# Autodesk Inventor assembly: XRevit Filter column D1200
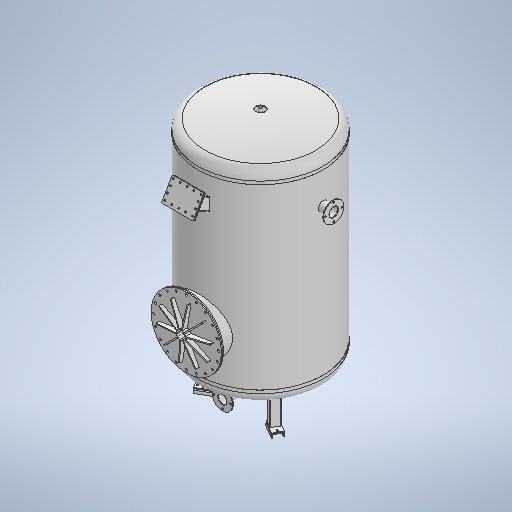
[picture p0: Inventor's stored thumbnail of the model, 512x512]
Saved by Autodesk Inventor 2025.4 (Build 294407000, 407)
## iProperties
Created: 2025-02-13
Part Number: XRevit Filter column D1200
Document SubType Name: Assembly
Designer: pokla
Mass: 483166 g
Surface Area: 236267 cm^2
Volume: 67816.7 cm^3
Density: 7.1246 g/cm^3
allow_slope_adjustment: 0 ul
flow_configuration2: 1 ul
flow_direction: 2 ul
loss_method: 0 ul
radius: 45,500 mm
radius: 16,750 mm
Author: pokla
Revision Number: 3
## Documents named in this file (23)
- C:\Users\pokla\Documents\Inventor\PRS-Purovskii\Model\PRS-filter 1200\ASY PRS Filter column D1200.iam
- C:\Users\pokla\Documents\Inventor\PRS-Purovskii\Model\PRS-filter 1200\PRS 1200-22 accses hatch flangeipt.ipt
- C:\Users\pokla\Documents\Inventor\PRS-Purovskii\Model\PRS-filter 1200\PRS 1200-11 accses hatch tube.ipt
- C:\Users\pokla\Documents\Inventor\PRS-Purovskii\Model\PRS-filter 1200\PRS 1200-02 dished head.ipt
- C:\Users\pokla\Documents\Inventor\PRS-Purovskii\Model\PRS-filter 1200\Fitting G1.ipt
- C:\Users\pokla\Documents\Inventor\PRS-Purovskii\Model\PRS-filter 1200\ASY PRS 1200-90 Filter legs.iam
- C:\Users\pokla\Documents\Inventor\PRS-Purovskii\Model\PRS-filter 1200\PRS 1200-33 charging blind flange.ipt
- C:\Users\pokla\Documents\Inventor\PRS-Purovskii\Model\PRS-filter 1200\ASY PRS 1200-20 charging hatch.iam
- C:\Users\pokla\Documents\Inventor\PRS-Purovskii\Model\PRS-filter 1200\PRS 1200-12 FDS tube 2.ipt
- C:\Users\pokla\Documents\Inventor\PRS-Purovskii\Model\PRS-filter 1200\PRS 1200-06 charging flange round.ipt
- C:\Users\pokla\Documents\Inventor\PRS-Purovskii\Model\PRS-filter 1200\PRS 1200-13 FDS tube 3.ipt
- C:\Users\pokla\Documents\Inventor\PRS-Purovskii\Model\PRS-filter 1200\PRS 1200-14 FDS tube 4.ipt
- C:\Users\pokla\Documents\Inventor\PRS-Purovskii\Model\PRS-filter 1200\PRS 1200-15 FDS tube 5.ipt
- C:\Users\pokla\Documents\Inventor\PRS-Purovskii\Model\PRS-filter 1200\PRS 1200-31 FDS flange DN90.ipt
- C:\Users\pokla\Documents\Inventor\PRS-Purovskii\Model\PRS-filter 1200\PRS 1200-32 FDS free flange DN90.ipt
- C:\Users\pokla\Documents\Inventor\PRS-Purovskii\Model\PRS-filter 1200\PRS 1200-71 charging tube 1.ipt
- C:\Users\pokla\Documents\Inventor\PRS-Purovskii\Model\PRS-filter 1200\PRS 1200-72 charging tube 2.ipt
- C:\Users\pokla\Documents\Inventor\PRS-Purovskii\Model\PRS-filter 1200\PRS 1200-07 charging flange rect.ipt
- C:\Users\pokla\Documents\Inventor\PRS-Purovskii\Model\PRS-filter 1200\PRS 1200-10 main Shell.ipt
- C:\Users\pokla\Documents\Inventor\PRS-Purovskii\Model\PRS-filter 1200\JIS B 2312 90 Deg Long Elbow Steel 50A x Sch 40.ipt
- C:\Users\pokla\Documents\Inventor\PRS-Purovskii\Model\PRS-filter 1200\ASY PRS 1200-80 top funnel .iam
- C:\Users\pokla\Documents\Inventor\PRS-Purovskii\Model\PRS-filter 1200\ASY PRS 1200-50 filter-distribution-system.iam
- C:\Users\pokla\Documents\Inventor\PRS-Purovskii\Model\PRS-filter 1200\JIS B 2312 90 Deg Long Elbow Steel 80A x Sch 40.ipt
## Components (28 placed, 23 different names)
1. Fitting G1.ipt:1 — Rigid:15
2. PNS 1633 charging blind flange.ipt:2 — Rigid:67
3. PRS 940-10 main Shell D 940:1 — Flush:7, Rigid:85, Flush:8, Rotational:76, Rotational:77, Rigid:86, Rigid:87
4. PRS 1200-33 charging blind flange:5 — Rigid:77
5. PRS 1200-33 charging blind flange:6 — Rigid:78, Rigid:90
6. PNS 1604 dished head D1000.ipt:1 — Rotational:77, Rigid:88, Mate:7
7. Fitting G1.ipt:2 — Mate:4, Mate:5, Mate:6
8. JIS B 2312 90 Deg Long Elbow Steel 80A x Sch 40.ipt:1 — Rigid:68, Rigid:79, Mate:6, Rigid:88
9. PRS 1200-13 FDS tube 3:1 — Rigid:67, Rigid:68, Flush:9
10. PRS 1200-14 FDS tube 4:1 — Rigid:79, Rotational:71
11. PRS 1200-31 FDS flange DN90:1 — Rigid:76
12. PRS 1200-32 FDS free flange DN90:1 — Rotational:71, Rigid:76, Rotational:78
13. PNS-611 accses hatch tube.ipt:1 — Rotational:74, Rigid:85
14. PNS 1604 dished head D1000.ipt:2 — Rigid:15, Rotational:76
15. JIS B 2312 90 Deg Long Elbow Steel 80A x Sch 40.ipt:2 — Rigid:62, Rigid:73
16. PRS 1200-12 FDS tube 2:3 — Rigid:62, Rigid:78
17. PRS 1200-15 FDS tube 5:1 — Rigid:73, Rigid:77, Rigid:87
18. PRS 1200-72 charging tube 2:1 — Rigid:84, Rigid:89
19. PRS 1200-71 charging tube 1:1 — Rigid:84, Rigid:86
20. PRS 940-06 charging flange round:1 — Rigid:83, Rigid:89
21. PRS 940-07 charging flange rect:1 — Rigid:83
22. PNS-612 accses hatch flangeipt.ipt:1 — Rotational:73, Rotational:74
23. ASY PNS 1610 charging hatch.iam:1 [sub-assembly] — Rotational:73
24. ASY PRS 1200-80  top funnel :1 [sub-assembly] — Rigid:90
25. ASY PRS 1200-50 filter-distribution-system:1 [sub-assembly] — Rotational:78
26. ASY PNS 1690 Filter legs D1000.iam:1 [sub-assembly] — Flush:2, Flush:10, Flush:11
27. ASY PRS 1200-90 Filter legs:2 [sub-assembly]
28. ASY PRS 1200-90 Filter legs:3 [sub-assembly]
## Component patterns: (3 elements, first: ASY PNS 1690 Filter legs D1000.iam:1)
## Relationships (33: WeldJoint 17, Flush 6, RevoluteJoint 6, Mate 4)
- Rigid:15 [WeldJoint]: Fitting G1.ipt:1 ↔ PNS 1604 dished head D1000.ipt:2
- Flush:2: ASY PNS 1690 Filter legs D1000.iam:1
- Rigid:62 [WeldJoint]: JIS B 2312 90 Deg Long Elbow Steel 80A x Sch 40.ipt:2 ↔ PRS 1200-12 FDS tube 2:3
- Rigid:67 [WeldJoint]: PNS 1633 charging blind flange.ipt:2 ↔ PRS 1200-13 FDS tube 3:1
- Rigid:68 [WeldJoint]: JIS B 2312 90 Deg Long Elbow Steel 80A x Sch 40.ipt:1 ↔ PRS 1200-13 FDS tube 3:1
- Rigid:79 [WeldJoint] (1 mm): JIS B 2312 90 Deg Long Elbow Steel 80A x Sch 40.ipt:1 ↔ PRS 1200-14 FDS tube 4:1
- Rigid:73 [WeldJoint]: JIS B 2312 90 Deg Long Elbow Steel 80A x Sch 40.ipt:2 ↔ PRS 1200-15 FDS tube 5:1
- Rotational:71 [RevoluteJoint]: PRS 1200-14 FDS tube 4:1 ↔ PRS 1200-32 FDS free flange DN90:1
- Rigid:76 [WeldJoint]: PRS 1200-31 FDS flange DN90:1 ↔ PRS 1200-32 FDS free flange DN90:1
- Rigid:77 [WeldJoint]: PRS 1200-33 charging blind flange:5 ↔ PRS 1200-15 FDS tube 5:1
- Rigid:78 [WeldJoint]: PRS 1200-33 charging blind flange:6 ↔ PRS 1200-12 FDS tube 2:3
- Rotational:73 [RevoluteJoint]: PNS-612 accses hatch flangeipt.ipt:1 ↔ ASY PNS 1610 charging hatch.iam:1
- Rotational:74 [RevoluteJoint]: PNS-611 accses hatch tube.ipt:1 ↔ PNS-612 accses hatch flangeipt.ipt:1
- Rigid:83 [WeldJoint]: PRS 940-06 charging flange round:1 ↔ PRS 940-07 charging flange rect:1
- Rigid:84 [WeldJoint]: PRS 1200-72 charging tube 2:1 ↔ PRS 1200-71 charging tube 1:1
- Flush:10: ASY PNS 1690 Filter legs D1000.iam:1
- Flush:11: ASY PNS 1690 Filter legs D1000.iam:1
- Flush:7: PRS 940-10 main Shell D 940:1
- Rigid:85 [WeldJoint]: PRS 940-10 main Shell D 940:1 ↔ PNS-611 accses hatch tube.ipt:1
- Flush:8: PRS 940-10 main Shell D 940:1
- Rotational:76 [RevoluteJoint]: PRS 940-10 main Shell D 940:1 ↔ PNS 1604 dished head D1000.ipt:2
- Rotational:77 [RevoluteJoint]: PRS 940-10 main Shell D 940:1 ↔ PNS 1604 dished head D1000.ipt:1
- Flush:9: PRS 1200-13 FDS tube 3:1
- Rigid:86 [WeldJoint]: PRS 940-10 main Shell D 940:1 ↔ PRS 1200-71 charging tube 1:1
- Rigid:87 [WeldJoint] (100 mm): PRS 940-10 main Shell D 940:1 ↔ PRS 1200-15 FDS tube 5:1
- Mate:4: Fitting G1.ipt:2
- Mate:5 (150 mm): Fitting G1.ipt:2
- Mate:6: Fitting G1.ipt:2 ↔ JIS B 2312 90 Deg Long Elbow Steel 80A x Sch 40.ipt:1
- Rigid:88 [WeldJoint] (1 mm): PNS 1604 dished head D1000.ipt:1 ↔ JIS B 2312 90 Deg Long Elbow Steel 80A x Sch 40.ipt:1
- Rigid:89 [WeldJoint]: PRS 1200-72 charging tube 2:1 ↔ PRS 940-06 charging flange round:1
- Rigid:90 [WeldJoint]: PRS 1200-33 charging blind flange:6 ↔ ASY PRS 1200-80  top funnel :1
- Rotational:78 [RevoluteJoint]: PRS 1200-32 FDS free flange DN90:1 ↔ ASY PRS 1200-50 filter-distribution-system:1
- Mate:7 (300 mm): PNS 1604 dished head D1000.ipt:1
